# Autodesk Inventor assembly: EstructuraInferior
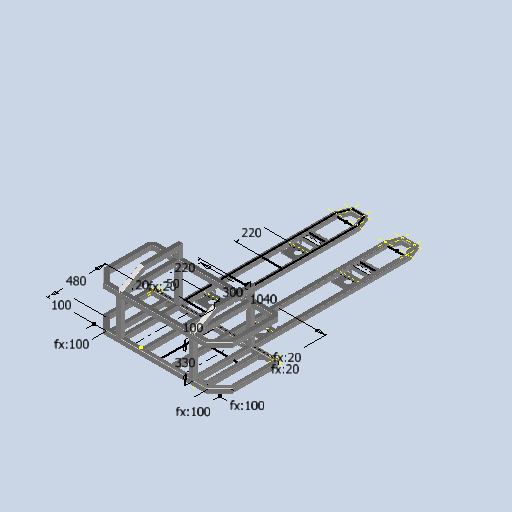
[picture p0: Inventor's stored thumbnail of the model, 512x512]
Saved by Autodesk Inventor 2022.1 (Build 261234000, 234)
## iProperties
Created: 2021-09-22
Part Number: EstructuraInferior
Material: Generic
Document SubType Name: Weldment
Designer: Andres
Mass: 82364 g
Surface Area: 55360.1 cm^2
Volume: 10500.9 cm^3
Density: 7.84348 g/cm^3
Weld Material: Steel, Alloy
_SolveAssemblyDoc: Frame Generator Solve Assembly
_Version: 25.0.0
Author: Andres
## Documents named in this file (11)
- C:\Users\seb_0\Desktop\PDM\ProyectoRobotPallet\Estructura Inferior\EstructuraInferior - Soldadura.iam
- C:\Users\seb_0\Desktop\PDM\ProyectoRobotPallet\Estructura Inferior\EstructuraInferior_Esqueleto.ipt
- C:\Users\seb_0\Desktop\PDM\ProyectoRobotPallet\Estructura Inferior\Frame_Base.iam
- C:\Users\seb_0\Desktop\PDM\ProyectoRobotPallet\HorquillaSuperior\HorquillaSuperior.ipt
- C:\Users\seb_0\Desktop\PDM\ProyectoRobotPallet\SistemaDeElevacion\version2\BaseSistema.ipt
- C:\Users\seb_0\Desktop\PDM\ProyectoRobotPallet\Estructura Inferior\EstructuraInferior - Soldadura\AIP\FEA\dr4lsv0ao.fins
- C:\Users\seb_0\Desktop\PDM\ProyectoRobotPallet\Estructura Inferior\EstructuraInferior - Soldadura\AIP\FEA\dr4lsv0ao.fsat
- C:\Users\seb_0\Desktop\PDM\ProyectoRobotPallet\Estructura Inferior\EstructuraInferior - Soldadura\AIP\FEA\dr4lsv0ao.ftes
- C:\Users\seb_0\Desktop\PDM\ProyectoRobotPallet\Estructura Inferior\EstructuraInferior - Soldadura\AIP\FEA\dr4lsv0ao.fwiz
- C:\Users\seb_0\Desktop\PDM\ProyectoRobotPallet\Estructura Inferior\EstructuraInferior - Soldadura\AIP\FEA\dr4lsv4bk.fmsh
- C:\Users\seb_0\Desktop\PDM\ProyectoRobotPallet\Estructura Inferior\EstructuraInferior - Soldadura\AIP\FEA\dr4lsv4bl.fres
## Components (7 placed, 4 different names)
1. EstructuraInferior_Esqueleto:1 — Mate:2, Mate:3, Mate:4, Mate:5, Mate:7, Mate:9, Mate:10, Mate:12
2. Frame_Base:1 [sub-assembly] — Flush:1, Mate:1, Mate:6, Mate:8, Mate:11
3. HorquillaSuperior:1 — Flush:1
4. BaseSistema:1 — Mate:1, Mate:2, Mate:3
5. BaseSistema:2 — Mate:10, Mate:11, Mate:12
6. BaseSistema:3 — Mate:4, Mate:5, Mate:6
7. BaseSistema:4 — Mate:7, Mate:8, Mate:9
## Relationships (13: Mate 12, Flush 1)
- Flush:1: Frame_Base:1 ↔ HorquillaSuperior:1
- Mate:1: Frame_Base:1 ↔ BaseSistema:1
- Mate:2: EstructuraInferior_Esqueleto:1 ↔ BaseSistema:1
- Mate:3: EstructuraInferior_Esqueleto:1 ↔ BaseSistema:1
- Mate:4: EstructuraInferior_Esqueleto:1 ↔ BaseSistema:3
- Mate:5: EstructuraInferior_Esqueleto:1 ↔ BaseSistema:3
- Mate:6: Frame_Base:1 ↔ BaseSistema:3
- Mate:7: EstructuraInferior_Esqueleto:1 ↔ BaseSistema:4
- Mate:8: Frame_Base:1 ↔ BaseSistema:4
- Mate:9: EstructuraInferior_Esqueleto:1 ↔ BaseSistema:4
- Mate:10: EstructuraInferior_Esqueleto:1 ↔ BaseSistema:2
- Mate:11: Frame_Base:1 ↔ BaseSistema:2
- Mate:12: EstructuraInferior_Esqueleto:1 ↔ BaseSistema:2
## Named parameters: sa_18 = 0, sa_19 = -250000, sa_20 = 0, sa_21 = 0, sa_22 = -250000, sa_23 = 0, sa_24 = 0, sa_25 = -250000, sa_26 = 0, sa_27 = 0, sa_28 = -250000, sa_29 = 0
note: some values were not read from the file. Shown as the stored number, unit unknown: "sa_18", "sa_19", "sa_20", "sa_21", "sa_22", "sa_23", "sa_24", "sa_25", "sa_26", "sa_27", "sa_28", "sa_29".
